# Autodesk Inventor assembly: LeftMecanumDTANewAttachment
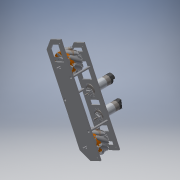
[picture p0: Inventor's stored thumbnail of the model, 180x180]
Saved by Autodesk Inventor 2017 (Build 210142000, 142)
## iProperties
Created: 2017-08-12
Part Number: LeftMecanumDTANewAttachment
Document SubType Name: Assembly
Designer: User
Author: User
## Documents named in this file (7)
- C:\Robotics\CAD\2016-17_CAD\DriveTrain\LeftMecanumDTANewAttachment.iam
- C:\Robotics\CAD\2016-17_CAD\DriveTrain\DrainTrainPlate2.0LeftOutside.iam
- C:\Robotics\CAD\2016-17_CAD\DriveTrain\DriveTrainPlate2.0LeftInside.ipt
- C:\Robotics\CAD\2016-17_CAD\DriveTrain\motor sub assembley.iam
- C:\Robotics\CAD\COTSParts\Tetrix\tetrix-motor-mounts-1.snapshot.1\Tetrex 2pc motor mount.ipt
- C:\Robotics\CAD\2016-17_CAD\DriveTrain\drive train standoff.0002.ipt
- C:\Robotics\CAD\2016-17_CAD\DriveTrain\NewMechanumWheelSubAssembly.iam
## Components (11 placed, 6 different names)
1. DrainTrainPlate2.0LeftOutside:1 [sub-assembly] — Mate:14, Mate:15, Mate:16, Mate:26, Mate:27
2. motor sub assembley:1 [sub-assembly] — Mate:13
3. motor sub assembley:2 [sub-assembly] — Mate:9
4. Tetrex 2pc motor mount:1 — Mate:9, Mate:23, Mate:24, Mate:25
5. Tetrex 2pc motor mount:2 — Mate:13, Mate:20, Mate:21, Mate:22
6. drive train standoff.0002:1 — Mate:14
7. drive train standoff.0002:2 — Mate:15
8. drive train standoff.0002:3 — Mate:16
9. DriveTrainPlate2.0LeftInside:1 — Mate:20, Mate:21, Mate:22, Mate:23, Mate:24, Mate:25, Flush:1, Flush:2, Mate:28, Mate:29, Mate:30
10. NewMechanumWheelSubAssembly:1 [sub-assembly] — Mate:26, Flush:1, Mate:29, Mate:30
11. NewMechanumWheelSubAssembly:2 [sub-assembly] — Mate:27, Flush:2, Mate:28
## Relationships (18: Mate 16, Flush 2)
- Mate:9: motor sub assembley:2 ↔ Tetrex 2pc motor mount:1
- Mate:13: motor sub assembley:1 ↔ Tetrex 2pc motor mount:2
- Mate:14: DrainTrainPlate2.0LeftOutside:1 ↔ drive train standoff.0002:1
- Mate:15: DrainTrainPlate2.0LeftOutside:1 ↔ drive train standoff.0002:2
- Mate:16: DrainTrainPlate2.0LeftOutside:1 ↔ drive train standoff.0002:3
- Mate:20: Tetrex 2pc motor mount:2 ↔ DriveTrainPlate2.0LeftInside:1
- Mate:21: Tetrex 2pc motor mount:2 ↔ DriveTrainPlate2.0LeftInside:1
- Mate:22: Tetrex 2pc motor mount:2 ↔ DriveTrainPlate2.0LeftInside:1
- Mate:23: Tetrex 2pc motor mount:1 ↔ DriveTrainPlate2.0LeftInside:1
- Mate:24: Tetrex 2pc motor mount:1 ↔ DriveTrainPlate2.0LeftInside:1
- Mate:25: Tetrex 2pc motor mount:1 ↔ DriveTrainPlate2.0LeftInside:1
- Mate:26: DrainTrainPlate2.0LeftOutside:1 ↔ NewMechanumWheelSubAssembly:1
- Flush:1: DriveTrainPlate2.0LeftInside:1 ↔ NewMechanumWheelSubAssembly:1
- Mate:27: DrainTrainPlate2.0LeftOutside:1 ↔ NewMechanumWheelSubAssembly:2
- Flush:2: DriveTrainPlate2.0LeftInside:1 ↔ NewMechanumWheelSubAssembly:2
- Mate:28: DriveTrainPlate2.0LeftInside:1 ↔ NewMechanumWheelSubAssembly:2
- Mate:29: DriveTrainPlate2.0LeftInside:1 ↔ NewMechanumWheelSubAssembly:1
- Mate:30 (6.35 mm): DriveTrainPlate2.0LeftInside:1 ↔ NewMechanumWheelSubAssembly:1
